# Autodesk Inventor assembly: DriveSide_6inchWheels_Options
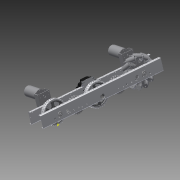
[picture p0: Inventor's stored thumbnail of the model, 180x180]
Saved by Autodesk Inventor 2015 (Build 190159000, 159)
## iProperties
Created: 2016-01-10
Part Number: DriveSide_6inchWheels_Options
Document SubType Name: Assembly
Designer: Applefamily
Author: Applefamily
## Documents named in this file (12)
- C:\Users\Applegate\Desktop\Chassy_Wheeled\Assembly\DriveSide_6inchWheels_Options.iam
- C:\Users\Applegate\Desktop\Chassy_Wheeled\Assembly\Imported Components\am-2951 AM14U2 Outside Sheet.ipt\am-2951 AM14U2 Outside Sheet.ipt.ipt
- C:\Users\Applegate\Desktop\Chassy_Wheeled\Assembly\GearBox and Mec.iam
- C:\Users\Applegate\Desktop\Chassy_Wheeled\Assembly\Imported Components\FR8ZZ Hex Bearing.ipt\FR8ZZ Hex Bearing.ipt.ipt
- C:\Users\Applegate\Desktop\Chassy_Wheeled\Assembly\Imported Components\am-2952 AM14U2 Inside Sheet.ipt\am-2952 AM14U2 Inside Sheet.ipt.ipt
- C:\Users\Applegate\Downloads\Imported Components\4 in HiGrip Wheel\4 in HiGrip Wheel.iam
- C:\Users\Applegate\Downloads\Imported Components\AM14U3+Long+REV1-1\am-2598_107 2016 KOP Toughbox Mini.iam
- C:\Users\Applegate\Desktop\Chassy_Wheeled\Assembly\GearBox and Grip.iam
- C:\Users\Applegate\Downloads\Imported Components\am-940a-6-HiGrip-\am-940a-6-HiGrip-.iam
- am-2951 AM14U2 Outside Sheet.ipt
- FR8ZZ Hex Bearing.ipt
- am-2952 AM14U2 Inside Sheet.ipt
## Components (10 placed, 8 different names)
1. am-2951 AM14U2 Outside Sheet.ipt:1 — Cylindrical:1, Cylindrical:2, Mate:1, Mate:2, Cylindrical:7, Cylindrical:8
2. FR8ZZ Hex Bearing.ipt:1 — Cylindrical:1, Mate:1
3. FR8ZZ Hex Bearing.ipt:2 — Cylindrical:2, Mate:2, Cylindrical:3
4. GearBox and Mec:2 [sub-assembly] — Cylindrical:3, Cylindrical:5, Mate:4
5. am-2952 AM14U2 Inside Sheet.ipt:1 — Cylindrical:5, Mate:4, Rotational:1, Rotational:2
6. 4 in HiGrip Wheel:2 [sub-assembly] — Flush:1, Cylindrical:8
7. 4 in HiGrip Wheel:3 [sub-assembly] — Flush:2, Flush:3, Cylindrical:7
8. am-2598_107 2016 KOP Toughbox Mini:1 [sub-assembly] — Rotational:1, Cylindrical:6
9. GearBox and Grip:1 [sub-assembly] — Rotational:2, Flush:3, Mate:5
10. am-940a-6-HiGrip-:1 [sub-assembly] — Cylindrical:6, Flush:1, Flush:2
## Relationships (16: CylindricalJoint 7, Mate 4, Flush 3, RevoluteJoint 2)
- Cylindrical:1: am-2951 AM14U2 Outside Sheet.ipt:1 ↔ FR8ZZ Hex Bearing.ipt:1
- Cylindrical:2: am-2951 AM14U2 Outside Sheet.ipt:1 ↔ FR8ZZ Hex Bearing.ipt:2
- Mate:1: am-2951 AM14U2 Outside Sheet.ipt:1 ↔ FR8ZZ Hex Bearing.ipt:1
- Mate:2: am-2951 AM14U2 Outside Sheet.ipt:1 ↔ FR8ZZ Hex Bearing.ipt:2
- Cylindrical:3: FR8ZZ Hex Bearing.ipt:2 ↔ GearBox and Mec:2
- Cylindrical:5: GearBox and Mec:2 ↔ am-2952 AM14U2 Inside Sheet.ipt:1
- Mate:4: GearBox and Mec:2 ↔ am-2952 AM14U2 Inside Sheet.ipt:1
- Rotational:1 [RevoluteJoint]: am-2952 AM14U2 Inside Sheet.ipt:1 ↔ am-2598_107 2016 KOP Toughbox Mini:1
- Rotational:2 [RevoluteJoint]: am-2952 AM14U2 Inside Sheet.ipt:1 ↔ GearBox and Grip:1
- Cylindrical:6: am-2598_107 2016 KOP Toughbox Mini:1 ↔ am-940a-6-HiGrip-:1
- Flush:1: 4 in HiGrip Wheel:2 ↔ am-940a-6-HiGrip-:1
- Flush:2: 4 in HiGrip Wheel:3 ↔ am-940a-6-HiGrip-:1
- Flush:3: 4 in HiGrip Wheel:3 ↔ GearBox and Grip:1
- Cylindrical:7: am-2951 AM14U2 Outside Sheet.ipt:1 ↔ 4 in HiGrip Wheel:3
- Cylindrical:8: am-2951 AM14U2 Outside Sheet.ipt:1 ↔ 4 in HiGrip Wheel:2
- Mate:5: GearBox and Grip:1
